# Autodesk Inventor assembly: Ribbon Cable Male 15Pin
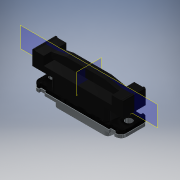
[picture p0: Inventor's stored thumbnail of the model, 180x180]
Saved by Autodesk Inventor 2019 (Build 230136000, 136)
## iProperties
Created: 2019-02-07
Part Number: Ribbon Cable Male 15Pin
Document SubType Name: Assembly
Designer: Serge
Author: Serge
## Documents named in this file (3)
- C:\Users\Serge\Desktop\Electrical\Parts\Ribbon Cable\Ribbon Cable Male 15Pin.iam
- C:\Users\Serge\Desktop\Electrical\Parts\Ribbon Cable\Dsub 15 Pin, 2 Row, Male.ipt
- C:\Users\Serge\Desktop\Electrical\Parts\Ribbon Cable\Ribbon mount 15Pin.ipt
## Components (2 placed, 2 different names)
1. Dsub 15 Pin, 2 Row, Male:1 — Mate:1, Flush:1, Flush:2
2. Ribbon mount 15Pin:1 — Mate:1, Flush:1, Flush:2
## Relationships (3: Flush 2, Mate 1)
- Mate:1: Dsub 15 Pin, 2 Row, Male:1 ↔ Ribbon mount 15Pin:1
- Flush:1: Dsub 15 Pin, 2 Row, Male:1 ↔ Ribbon mount 15Pin:1
- Flush:2: Dsub 15 Pin, 2 Row, Male:1 ↔ Ribbon mount 15Pin:1
